# Autodesk Inventor assembly: SubAssembly Undercarriage
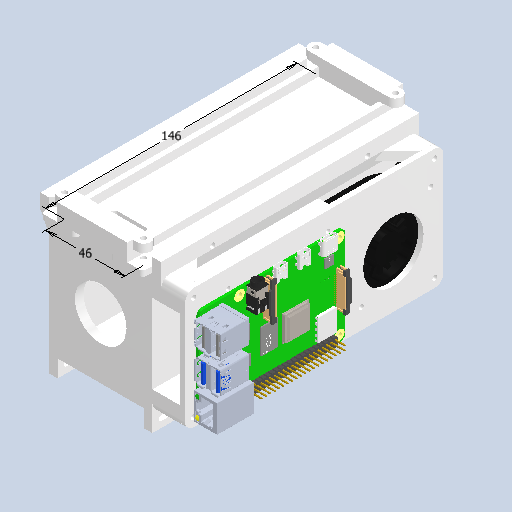
[picture p0: Inventor's stored thumbnail of the model, 512x512]
Saved by Autodesk Inventor 2023 (Build 270158000, 158)
## iProperties
Created: 2023-01-18
Part Number: SubAssembly Undercarriage
Document SubType Name: Assembly
Designer: Administrator
Author: Administrator
## Documents named in this file (6)
- C:\Users\chase\OneDrive\Documents\GitHub\WU-Team20-AutonomousDrone\CAD\ASSEMBLY\SubAssembly - BatteryCarrier WithAccessories.iam
- C:\Users\chase\OneDrive\Documents\GitHub\WU-Team20-AutonomousDrone\CAD\Electronics Mounts\BatteryCarrier - SlidingPlate Main.ipt
- C:\Users\chase\OneDrive\Documents\GitHub\WU-Team20-AutonomousDrone\CAD\Raw Models\BlowerFan.ipt
- C:\Users\chase\OneDrive\Documents\GitHub\WU-Team20-AutonomousDrone\CAD\Electronics Mounts\ChargingCircuit - ShroudPlate.ipt
- C:\Users\chase\OneDrive\Documents\GitHub\WU-Team20-AutonomousDrone\CAD\Electronics Mounts\BatteryCarrier - SlidingPlate ToothedMount.ipt
- C:\Users\chase\OneDrive\Documents\GitHub\WU-Team20-AutonomousDrone\CAD\Raw Models\Raspberry Pi Model 4B\Raspberry Pi 4 Model B.iam
## Components (5 placed, 5 different names)
1. BatteryCarrier - SlidingPlate Main:1 — Rigid:3, Mate:3, Flush:1, Mate:4
2. BlowerFan:1 — Mate:1, Mate:2
3. ChargingCircuit - ShroudPlate:1 — Mate:1, Mate:2, Rigid:3, Rigid:4
4. BatteryCarrier - SlidingPlate ToothedMount:1 — Mate:3, Flush:1, Mate:4
5. Raspberry Pi 4 Model B:1 [sub-assembly] — Rigid:4
## Relationships (7: Mate 4, WeldJoint 2, Flush 1)
- Mate:1: BlowerFan:1 ↔ ChargingCircuit - ShroudPlate:1
- Mate:2: BlowerFan:1 ↔ ChargingCircuit - ShroudPlate:1
- Rigid:3 [WeldJoint]: BatteryCarrier - SlidingPlate Main:1 ↔ ChargingCircuit - ShroudPlate:1
- Mate:3 (0.25 mm): BatteryCarrier - SlidingPlate Main:1 ↔ BatteryCarrier - SlidingPlate ToothedMount:1
- Flush:1 (-5 mm): BatteryCarrier - SlidingPlate Main:1 ↔ BatteryCarrier - SlidingPlate ToothedMount:1
- Mate:4 (0.5 mm): BatteryCarrier - SlidingPlate Main:1 ↔ BatteryCarrier - SlidingPlate ToothedMount:1
- Rigid:4 [WeldJoint] (5 mm): ChargingCircuit - ShroudPlate:1 ↔ Raspberry Pi 4 Model B:1
